# Autodesk Inventor assembly: 部件1
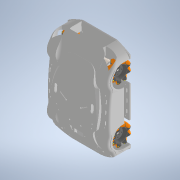
[picture p0: Inventor's stored thumbnail of the model, 180x180]
Saved by Autodesk Inventor 2020.3 (Build 243373000, 373)
## iProperties
Created: 2020-12-02
Part Number: 部件1
Document SubType Name: Assembly
Designer: huang
Author: huang
## Documents named in this file (6)
- D:\学校\小车\新建文件夹 (2)\知能ロボコン\部件2.iam
- D:\学校\小车\新建文件夹 (2)\知能ロボコン\底板2.ipt
- D:\学校\小车\新建文件夹 (2)\知能ロボコン\马达固定.ipt
- D:\学校\小车\新建文件夹 (2)\知能ロボコン\Moteur DC encodeur\Moteur DC encodeur.iam
- D:\学校\小车\新建文件夹 (2)\知能ロボコン\底板1.ipt
- D:\学校\小车\新建文件夹 (2)\知能ロボコン\3英寸麦轮.ipt
## Components (14 placed, 5 different names)
1. 底板2:1 — 插入:1, 插入:2, 插入:3, 插入:4, 插入:5, 插入:6, 插入:7, 插入:8, 插入:37
2. 马达固定:1 — 插入:1, 插入:2, 插入:25, 插入:26
3. 马达固定:2 — 插入:3, 插入:4, 插入:27, 插入:28
4. 马达固定:3 — 插入:5, 插入:6, 插入:21, 插入:22
5. 马达固定:4 — 插入:7, 插入:8, 插入:23, 插入:24
6. Moteur DC encodeur:1 [sub-assembly] — 插入:27, 插入:28, 插入:33
7. Moteur DC encodeur:2 [sub-assembly] — 插入:25, 插入:26, 插入:34
8. Moteur DC encodeur:3 [sub-assembly] — 插入:21, 插入:22, 插入:31
9. Moteur DC encodeur:4 [sub-assembly] — 插入:23, 插入:24, 插入:35
10. 底板1:1 — 插入:37
11. 3英寸麦轮:1 — 插入:31
12. 3英寸麦轮:2 — 插入:33
13. 3英寸麦轮:3 — 插入:34
14. 3英寸麦轮:4 — 插入:35
## Relationships (21: Insert 21)
- 插入:1 [Insert]: 底板2:1 ↔ 马达固定:1
- 插入:2 [Insert]: 底板2:1 ↔ 马达固定:1
- 插入:3 [Insert]: 底板2:1 ↔ 马达固定:2
- 插入:4 [Insert]: 底板2:1 ↔ 马达固定:2
- 插入:5 [Insert]: 底板2:1 ↔ 马达固定:3
- 插入:6 [Insert]: 底板2:1 ↔ 马达固定:3
- 插入:7 [Insert]: 底板2:1 ↔ 马达固定:4
- 插入:8 [Insert]: 底板2:1 ↔ 马达固定:4
- 插入:21 [Insert]: 马达固定:3 ↔ Moteur DC encodeur:3
- 插入:22 [Insert]: 马达固定:3 ↔ Moteur DC encodeur:3
- 插入:23 [Insert]: 马达固定:4 ↔ Moteur DC encodeur:4
- 插入:24 [Insert]: 马达固定:4 ↔ Moteur DC encodeur:4
- 插入:25 [Insert]: 马达固定:1 ↔ Moteur DC encodeur:2
- 插入:26 [Insert]: 马达固定:1 ↔ Moteur DC encodeur:2
- 插入:27 [Insert]: 马达固定:2 ↔ Moteur DC encodeur:1
- 插入:28 [Insert]: 马达固定:2 ↔ Moteur DC encodeur:1
- 插入:31 [Insert]: Moteur DC encodeur:3 ↔ 3英寸麦轮:1
- 插入:33 [Insert]: Moteur DC encodeur:1 ↔ 3英寸麦轮:2
- 插入:34 [Insert]: Moteur DC encodeur:2 ↔ 3英寸麦轮:3
- 插入:35 [Insert]: Moteur DC encodeur:4 ↔ 3英寸麦轮:4
- 插入:37 [Insert]: 底板2:1 ↔ 底板1:1
